# Autodesk Inventor assembly: slide with inserts_MIR
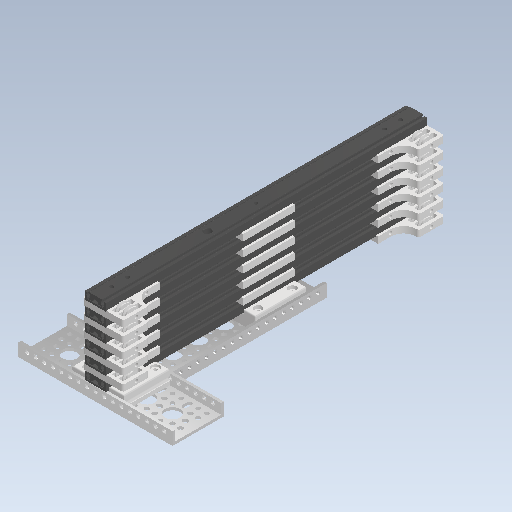
[picture p0: Inventor's stored thumbnail of the model, 512x512]
Saved by Autodesk Inventor 2020 (Build 240168000, 168)
## iProperties
Created: 2019-12-18
Part Number: slide with inserts_MIR
Document SubType Name: Assembly
Designer: xj82b
Author: xj82b
## Documents named in this file (8)
- C:\Users\xj82b\Documents\Inventor\5199\slide with inserts_MIR.iam
- C:\Users\xj82b\Documents\Inventor\5199\rightInsertbearings_MIR.iam
- C:\Users\xj82b\Documents\Inventor\5199\8x20x300mm-v2_MIR.ipt
- C:\Users\xj82b\Documents\Inventor\5199\leftInsertbearing_MIR.iam
- C:\Users\xj82b\Documents\Inventor\5199\centershortNEW_MIR.ipt
- C:\Users\xj82b\Documents\Inventor\5199\slidesmount_MIR.ipt
- C:\Users\xj82b\Documents\Inventor\5199\slidescentermount_MIR.ipt
- C:\Users\xj82b\Documents\Inventor\5199\gobilda parts\1121-0005-0144_MIR.ipt
## Components (26 placed, 7 different names)
1. rightInsertbearings_MIR:1 [sub-assembly] — Mate:53, Flush:26, Mate:52
2. 8x20x300mm-v2_MIR:1 — Mate:53, Flush:26, Mate:52, Mate:55, Flush:27, Mate:54, Mate:58, Mate:57, Mate:56, Flush:31, Mate:66, Flush:39, Flush:38
3. leftInsertbearing_MIR:1 [sub-assembly] — Mate:55, Flush:27, Mate:54, Flush:30
4. centershortNEW_MIR:1 — Mate:58, Mate:57, Mate:56, Mate:82
5. rightInsertbearings_MIR:2 [sub-assembly] — Mate:60, Flush:28, Mate:59
6. 8x20x300mm-v2_MIR:2 — Flush:31, Mate:60, Flush:28, Mate:59, Mate:62, Flush:29, Mate:61, Mate:64, Mate:65, Mate:63, Flush:47, Flush:46, Mate:98
7. leftInsertbearing_MIR:2 [sub-assembly] — Flush:30, Mate:62, Flush:29, Mate:61
8. centershortNEW_MIR:2 — Mate:66, Mate:64, Mate:65, Mate:63
9. 8x20x300mm-v2_MIR:3 — Mate:70, Flush:33, Mate:69, Flush:37, Mate:81, Mate:100, Flush:48, Mate:99, Mate:103, Mate:102, Mate:101
10. leftInsertbearing_MIR:3 [sub-assembly] — Mate:70, Flush:33, Mate:69, Flush:36
11. rightInsertbearings_MIR:3 [sub-assembly] — Mate:75, Flush:34, Mate:74
12. 8x20x300mm-v2_MIR:4 — Flush:39, Flush:38, Mate:82, Mate:75, Flush:34, Mate:74, Flush:37, Mate:77, Flush:35, Mate:76, Mate:79, Mate:80, Mate:78
13. leftInsertbearing_MIR:4 [sub-assembly] — Mate:77, Flush:36, Flush:35, Mate:76
14. centershortNEW_MIR:3 — Mate:79, Mate:81, Mate:80, Mate:78
15. rightInsertbearings_MIR:4 [sub-assembly] — Mate:84, Flush:40, Mate:83
16. 8x20x300mm-v2_MIR:5 — Flush:47, Flush:46, Mate:84, Flush:40, Mate:83, Mate:86, Flush:41, Mate:85, Mate:88, Mate:89, Mate:87, Flush:45, Mate:97
17. leftInsertbearing_MIR:5 [sub-assembly] — Mate:86, Flush:41, Mate:85, Flush:44
18. centershortNEW_MIR:4 — Mate:98, Mate:88, Mate:89, Mate:87
19. rightInsertbearings_MIR:5 [sub-assembly] — Mate:91, Flush:42, Mate:90
20. 8x20x300mm-v2_MIR:6 — Mate:91, Flush:42, Mate:90, Flush:45, Mate:93, Flush:43, Mate:92, Mate:95, Mate:96, Mate:94
21. leftInsertbearing_MIR:6 [sub-assembly] — Mate:93, Flush:44, Flush:43, Mate:92
22. centershortNEW_MIR:5 — Mate:95, Mate:97, Mate:96, Mate:94
23. slidesmount_MIR:1 — Mate:100, Flush:48, Mate:99, Flush:49, Mate:106, Mate:105, Mate:104
24. slidescentermount_MIR:1 — Flush:49, Mate:103, Mate:102, Mate:101, Mate:108, Mate:107
25. 1121-0005-0144_MIR:1 — Mate:108, Mate:107, Mate:109
26. 1121-0005-0144_MIR:2 — Mate:109, Mate:106, Mate:105, Mate:104
## Relationships (76: Mate 53, Flush 23)
- Mate:53: rightInsertbearings_MIR:1 ↔ 8x20x300mm-v2_MIR:1
- Flush:26: rightInsertbearings_MIR:1 ↔ 8x20x300mm-v2_MIR:1
- Mate:52: rightInsertbearings_MIR:1 ↔ 8x20x300mm-v2_MIR:1
- Mate:55: 8x20x300mm-v2_MIR:1 ↔ leftInsertbearing_MIR:1
- Flush:27: 8x20x300mm-v2_MIR:1 ↔ leftInsertbearing_MIR:1
- Mate:54: 8x20x300mm-v2_MIR:1 ↔ leftInsertbearing_MIR:1
- Mate:58: 8x20x300mm-v2_MIR:1 ↔ centershortNEW_MIR:1
- Mate:57: 8x20x300mm-v2_MIR:1 ↔ centershortNEW_MIR:1
- Mate:56: 8x20x300mm-v2_MIR:1 ↔ centershortNEW_MIR:1
- Flush:31: 8x20x300mm-v2_MIR:1 ↔ 8x20x300mm-v2_MIR:2
- Mate:60: rightInsertbearings_MIR:2 ↔ 8x20x300mm-v2_MIR:2
- Flush:28: rightInsertbearings_MIR:2 ↔ 8x20x300mm-v2_MIR:2
- Mate:59: rightInsertbearings_MIR:2 ↔ 8x20x300mm-v2_MIR:2
- Flush:30: leftInsertbearing_MIR:1 ↔ leftInsertbearing_MIR:2
- Mate:62: 8x20x300mm-v2_MIR:2 ↔ leftInsertbearing_MIR:2
- Flush:29: 8x20x300mm-v2_MIR:2 ↔ leftInsertbearing_MIR:2
- Mate:61: 8x20x300mm-v2_MIR:2 ↔ leftInsertbearing_MIR:2
- Mate:66: 8x20x300mm-v2_MIR:1 ↔ centershortNEW_MIR:2
- Mate:64: 8x20x300mm-v2_MIR:2 ↔ centershortNEW_MIR:2
- Mate:65: 8x20x300mm-v2_MIR:2 ↔ centershortNEW_MIR:2
- Mate:63: 8x20x300mm-v2_MIR:2 ↔ centershortNEW_MIR:2
- Mate:70: 8x20x300mm-v2_MIR:3 ↔ leftInsertbearing_MIR:3
- Flush:33: 8x20x300mm-v2_MIR:3 ↔ leftInsertbearing_MIR:3
- Mate:69: 8x20x300mm-v2_MIR:3 ↔ leftInsertbearing_MIR:3
- Flush:39: 8x20x300mm-v2_MIR:1 ↔ 8x20x300mm-v2_MIR:4
- Flush:38: 8x20x300mm-v2_MIR:1 ↔ 8x20x300mm-v2_MIR:4
- Mate:82: centershortNEW_MIR:1 ↔ 8x20x300mm-v2_MIR:4
- Mate:75: rightInsertbearings_MIR:3 ↔ 8x20x300mm-v2_MIR:4
- Flush:34: rightInsertbearings_MIR:3 ↔ 8x20x300mm-v2_MIR:4
- Mate:74: rightInsertbearings_MIR:3 ↔ 8x20x300mm-v2_MIR:4
- Flush:37: 8x20x300mm-v2_MIR:3 ↔ 8x20x300mm-v2_MIR:4
- Mate:77: 8x20x300mm-v2_MIR:4 ↔ leftInsertbearing_MIR:4
- Flush:36: leftInsertbearing_MIR:3 ↔ leftInsertbearing_MIR:4
- Flush:35: 8x20x300mm-v2_MIR:4 ↔ leftInsertbearing_MIR:4
- Mate:76: 8x20x300mm-v2_MIR:4 ↔ leftInsertbearing_MIR:4
- Mate:79: 8x20x300mm-v2_MIR:4 ↔ centershortNEW_MIR:3
- Mate:81: 8x20x300mm-v2_MIR:3 ↔ centershortNEW_MIR:3
- Mate:80: 8x20x300mm-v2_MIR:4 ↔ centershortNEW_MIR:3
- Mate:78: 8x20x300mm-v2_MIR:4 ↔ centershortNEW_MIR:3
- Flush:47: 8x20x300mm-v2_MIR:2 ↔ 8x20x300mm-v2_MIR:5
- Flush:46: 8x20x300mm-v2_MIR:2 ↔ 8x20x300mm-v2_MIR:5
- Mate:84: rightInsertbearings_MIR:4 ↔ 8x20x300mm-v2_MIR:5
- Flush:40: rightInsertbearings_MIR:4 ↔ 8x20x300mm-v2_MIR:5
- Mate:83: rightInsertbearings_MIR:4 ↔ 8x20x300mm-v2_MIR:5
- Mate:86: 8x20x300mm-v2_MIR:5 ↔ leftInsertbearing_MIR:5
- Flush:41: 8x20x300mm-v2_MIR:5 ↔ leftInsertbearing_MIR:5
- Mate:85: 8x20x300mm-v2_MIR:5 ↔ leftInsertbearing_MIR:5
- Mate:98: 8x20x300mm-v2_MIR:2 ↔ centershortNEW_MIR:4
- Mate:88: 8x20x300mm-v2_MIR:5 ↔ centershortNEW_MIR:4
- Mate:89: 8x20x300mm-v2_MIR:5 ↔ centershortNEW_MIR:4
- Mate:87: 8x20x300mm-v2_MIR:5 ↔ centershortNEW_MIR:4
- Mate:91: rightInsertbearings_MIR:5 ↔ 8x20x300mm-v2_MIR:6
- Flush:42: rightInsertbearings_MIR:5 ↔ 8x20x300mm-v2_MIR:6
- Mate:90: rightInsertbearings_MIR:5 ↔ 8x20x300mm-v2_MIR:6
- Flush:45: 8x20x300mm-v2_MIR:5 ↔ 8x20x300mm-v2_MIR:6
- Mate:93: 8x20x300mm-v2_MIR:6 ↔ leftInsertbearing_MIR:6
- Flush:44: leftInsertbearing_MIR:5 ↔ leftInsertbearing_MIR:6
- Flush:43: 8x20x300mm-v2_MIR:6 ↔ leftInsertbearing_MIR:6
- Mate:92: 8x20x300mm-v2_MIR:6 ↔ leftInsertbearing_MIR:6
- Mate:95: 8x20x300mm-v2_MIR:6 ↔ centershortNEW_MIR:5
- Mate:97: 8x20x300mm-v2_MIR:5 ↔ centershortNEW_MIR:5
- Mate:96: 8x20x300mm-v2_MIR:6 ↔ centershortNEW_MIR:5
- Mate:94: 8x20x300mm-v2_MIR:6 ↔ centershortNEW_MIR:5
- Mate:100: 8x20x300mm-v2_MIR:3 ↔ slidesmount_MIR:1
- Flush:48 (2.5 mm): 8x20x300mm-v2_MIR:3 ↔ slidesmount_MIR:1
- Mate:99: 8x20x300mm-v2_MIR:3 ↔ slidesmount_MIR:1
- Flush:49: slidesmount_MIR:1 ↔ slidescentermount_MIR:1
- Mate:103: 8x20x300mm-v2_MIR:3 ↔ slidescentermount_MIR:1
- Mate:102: 8x20x300mm-v2_MIR:3 ↔ slidescentermount_MIR:1
- Mate:101: 8x20x300mm-v2_MIR:3 ↔ slidescentermount_MIR:1
- Mate:108: slidescentermount_MIR:1 ↔ 1121-0005-0144_MIR:1
- Mate:107: slidescentermount_MIR:1 ↔ 1121-0005-0144_MIR:1
- Mate:109: 1121-0005-0144_MIR:1 ↔ 1121-0005-0144_MIR:2
- Mate:106: slidesmount_MIR:1 ↔ 1121-0005-0144_MIR:2
- Mate:105: slidesmount_MIR:1 ↔ 1121-0005-0144_MIR:2
- Mate:104: slidesmount_MIR:1 ↔ 1121-0005-0144_MIR:2
